# Autodesk Inventor assembly: case
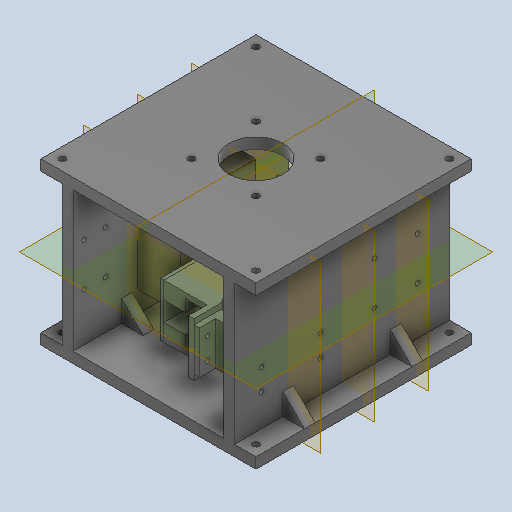
[picture p0: Inventor's stored thumbnail of the model, 512x512]
Saved by Autodesk Inventor 2026.2 (Build 302298010, 298A)
## iProperties
Created: 2026-05-01
Part Number: case
Document SubType Name: Assembly
Designer: chris
Author: chris
## Documents named in this file (9)
- C:\Users\chanh\내 드라이브\교과공부\2026년 1학기 (4학년 1학기)\01창의제품설계\CLOSE_hardware\04그리퍼\acrilic\case\case.iam
- C:\Users\chanh\내 드라이브\교과공부\2026년 1학기 (4학년 1학기)\01창의제품설계\CLOSE_hardware\04그리퍼\acrilic\case\main_case.ipt
- C:\Users\chanh\내 드라이브\교과공부\2026년 1학기 (4학년 1학기)\01창의제품설계\CLOSE_hardware\04그리퍼\acrilic\case\motor_bracket.ipt
- C:\Users\chanh\내 드라이브\교과공부\2026년 1학기 (4학년 1학기)\01창의제품설계\CLOSE_hardware\04그리퍼\acrilic\case\HTD-45H.ipt
- C:\Users\chanh\내 드라이브\교과공부\2026년 1학기 (4학년 1학기)\01창의제품설계\CLOSE_hardware\04그리퍼\acrilic\case\Top Horn.ipt
- C:\Users\chanh\내 드라이브\교과공부\2026년 1학기 (4학년 1학기)\01창의제품설계\CLOSE_hardware\04그리퍼\acrilic\case\pump.ipt
- C:\Users\chanh\내 드라이브\교과공부\2026년 1학기 (4학년 1학기)\01창의제품설계\CLOSE_hardware\04그리퍼\acrilic\case\nozzle_bracket.ipt
- C:\Users\chanh\내 드라이브\교과공부\2026년 1학기 (4학년 1학기)\01창의제품설계\CLOSE_hardware\04그리퍼\acrilic\case\nozzle_case.ipt
- C:\Users\chanh\내 드라이브\교과공부\2026년 1학기 (4학년 1학기)\01창의제품설계\CLOSE_hardware\04그리퍼\acrilic\case\nozzle_motor_bracket.ipt
## Components (8 placed, 8 different names)
1. main_case:1 — Flush:1, Flush:2, Flush:3, Mate:3, Mate:7, Mate:8, Flush:4, Mate:12, Mate:13
2. motor_bracket:1 — Mate:3, Mate:4, Mate:5, Mate:6, Mate:9, Mate:10, Mate:11, Mate:12, Mate:13
3. HTD-45H:1 — Mate:4, Mate:5, Mate:6, Insert:1
4. Top Horn:1 — Insert:1, Insert:2
5. pump:1 — Mate:7, Mate:8, Flush:4
6. nozzle_bracket:1 — Mate:9, Mate:10, Mate:11, Mate:14, Mate:15, Mate:16
7. nozzle_case:1 — Mate:14, Mate:15, Mate:16
8. nozzle_motor_bracket:1 — Insert:2
## Relationships (20: Mate 14, Flush 4, Insert 2)
- Flush:1: main_case:1
- Flush:2: main_case:1
- Flush:3: main_case:1
- Mate:3: main_case:1 ↔ motor_bracket:1
- Mate:4: motor_bracket:1 ↔ HTD-45H:1
- Mate:5: motor_bracket:1 ↔ HTD-45H:1
- Mate:6: motor_bracket:1 ↔ HTD-45H:1
- Insert:1: HTD-45H:1 ↔ Top Horn:1
- Mate:7: main_case:1 ↔ pump:1
- Mate:8 (20 mm): main_case:1 ↔ pump:1
- Flush:4 (70 mm): main_case:1 ↔ pump:1
- Mate:9: motor_bracket:1 ↔ nozzle_bracket:1
- Mate:10: motor_bracket:1 ↔ nozzle_bracket:1
- Mate:11: motor_bracket:1 ↔ nozzle_bracket:1
- Mate:12: main_case:1 ↔ motor_bracket:1
- Mate:13: main_case:1 ↔ motor_bracket:1
- Mate:14: nozzle_bracket:1 ↔ nozzle_case:1
- Mate:15: nozzle_bracket:1 ↔ nozzle_case:1
- Mate:16: nozzle_bracket:1 ↔ nozzle_case:1
- Insert:2: Top Horn:1 ↔ nozzle_motor_bracket:1
